# Autodesk Inventor assembly: byk_alternator
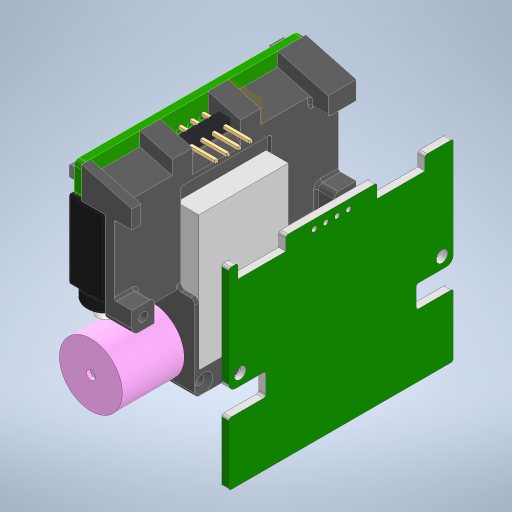
[picture p0: Inventor's stored thumbnail of the model, 512x512]
Saved by Autodesk Inventor 2023 (Build 270158000, 158)
## iProperties
Created: 2023-12-19
Part Number: byk_alternator
Document SubType Name: Assembly
Designer: Kamil
Author: Kamil
## Documents named in this file (12)
- C:\Users\Kamil\Documents\Inventor\MikroNalesnik\byk_alternator.iam
- C:\Users\Kamil\Documents\Inventor\MikroNalesnik\servo_mini_1370hd_cos.ipt
- C:\Users\Kamil\Documents\Inventor\MikroNalesnik\podstawa.ipt
- C:\Users\Kamil\Documents\Inventor\MikroNalesnik\noz2.ipt
- C:\Users\Kamil\Documents\Inventor\MikroNalesnik\QRE1113GR.ipt
- C:\Users\Kamil\Documents\Inventor\MikroNalesnik\silnik_2.ipt
- C:\Users\Kamil\Documents\Inventor\MikroNalesnik\kolko.ipt
- C:\Users\Kamil\Documents\Inventor\MikroNalesnik\pcb_dolne.ipt
- C:\Users\Kamil\Documents\Inventor\MikroNalesnik\4x_Male_Pin_2.54_mm.ipt
- C:\Users\Kamil\Documents\Inventor\MikroNalesnik\30x20x5.ipt
- C:\Users\Kamil\Desktop\MikroSumo.ipt
- C:\Users\Kamil\Documents\Inventor\MikroNalesnik\PCB_GORNE.ipt
## Components (15 placed, 11 different names)
1. servo_mini_1370hd_cos:1 — Zestawiające:1, Równoległe:1, Równoległe:2
2. servo_mini_1370hd_cos:2 — Zestawiające:1, Równoległe:1, Równoległe:2, Równoległe:3
3. podstawa:1 — Równoległe:3, Równoległe:4, Zestawiające:11, Równoległe:5, Równoległe:6, Zestawiające:17, Zestawiające:18, Zestawiające:19, Równoległe:7, Zestawiające:20, Zestawiające:38, Zestawiające:39, Zestawiające:40, Zestawiające:41, Zestawiające:42, Zestawiające:43, Równoległe:8, Zestawiające:44, Zestawiające:46, Zestawiające:47, Zestawiające:48
4. noz2:1 — Równoległe:4
5. QRE1113GR:1 — Zestawiające:18
6. QRE1113GR:2 — Zestawiające:17
7. silnik_2:1 — Zestawiające:11, Zestawiające:12, Zestawiające:13, Zestawiające:16
8. silnik_2:2 — Zestawiające:12, Zestawiające:13, Zestawiające:14, Zestawiające:15
9. kolko:1 — Zestawiające:14, Zestawiające:15, Równoległe:5
10. kolko:2 — Równoległe:6, Zestawiające:16
11. pcb_dolne:1 — Zestawiające:19, Równoległe:7, Zestawiające:20, Zestawiające:37
12. 4x_Male_Pin_2.54_mm:1 — Zestawiające:37
13. 30x20x5:1 — Zestawiające:38, Zestawiające:39, Zestawiające:46, Zestawiające:47, Zestawiające:48
14. MikroSumo:1 — Zestawiające:40, Zestawiające:41, Zestawiające:42
15. PCB_GORNE:1 — Zestawiające:43, Równoległe:8, Zestawiające:44
## Relationships (30: Mate 22, Flush 8)
- Zestawiające:1 [Mate] (-50 mm): servo_mini_1370hd_cos:1 ↔ servo_mini_1370hd_cos:2
- Równoległe:1 [Flush]: servo_mini_1370hd_cos:1 ↔ servo_mini_1370hd_cos:2
- Równoległe:2 [Flush]: servo_mini_1370hd_cos:1 ↔ servo_mini_1370hd_cos:2
- Równoległe:3 [Flush]: servo_mini_1370hd_cos:2 ↔ podstawa:1
- Równoległe:4 [Flush]: podstawa:1 ↔ noz2:1
- Zestawiające:11 [Mate]: podstawa:1 ↔ silnik_2:1
- Zestawiające:12 [Mate] (2 mm): silnik_2:1 ↔ silnik_2:2
- Zestawiające:13 [Mate]: silnik_2:1 ↔ silnik_2:2
- Zestawiające:14 [Mate]: silnik_2:2 ↔ kolko:1
- Zestawiające:15 [Mate]: silnik_2:2 ↔ kolko:1
- Równoległe:5 [Flush]: podstawa:1 ↔ kolko:1
- Równoległe:6 [Flush]: podstawa:1 ↔ kolko:2
- Zestawiające:16 [Mate]: silnik_2:1 ↔ kolko:2
- Zestawiające:17 [Mate] (1.6 mm): podstawa:1 ↔ QRE1113GR:2
- Zestawiające:18 [Mate] (1.6 mm): podstawa:1 ↔ QRE1113GR:1
- Zestawiające:19 [Mate]: podstawa:1 ↔ pcb_dolne:1
- Równoległe:7 [Flush]: podstawa:1 ↔ pcb_dolne:1
- Zestawiające:20 [Mate]: podstawa:1 ↔ pcb_dolne:1
- Zestawiające:37 [Mate]: pcb_dolne:1 ↔ 4x_Male_Pin_2.54_mm:1
- Zestawiające:38 [Mate]: podstawa:1 ↔ 30x20x5:1
- Zestawiające:39 [Mate] (0.1 mm): podstawa:1 ↔ 30x20x5:1
- Zestawiające:40 [Mate]: podstawa:1 ↔ MikroSumo:1
- Zestawiające:41 [Mate]: podstawa:1 ↔ MikroSumo:1
- Zestawiające:42 [Mate]: podstawa:1 ↔ MikroSumo:1
- Zestawiające:43 [Mate] (20 mm): podstawa:1 ↔ PCB_GORNE:1
- Równoległe:8 [Flush]: podstawa:1 ↔ PCB_GORNE:1
- Zestawiające:44 [Mate]: podstawa:1 ↔ PCB_GORNE:1
- Zestawiające:46 [Mate]: podstawa:1 ↔ 30x20x5:1
- Zestawiające:47 [Mate]: podstawa:1 ↔ 30x20x5:1
- Zestawiające:48 [Mate]: podstawa:1 ↔ 30x20x5:1
